# Autodesk Inventor assembly: omniwheelassmebly
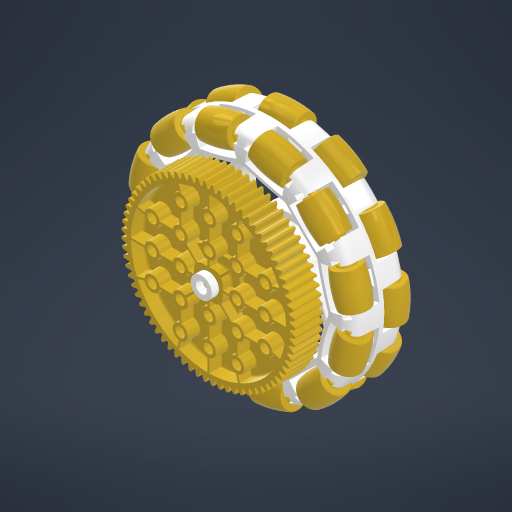
[picture p0: Inventor's stored thumbnail of the model, 512x512]
Saved by Autodesk Inventor 2023 (Build 270158000, 158)
## iProperties
Created: 2023-08-05
Part Number: omniwheelassmebly
Document SubType Name: Assembly
Designer: srbel
Author: srbel
## Documents named in this file (11)
- C:\CAD\OverUnderCAD\Drive\omniwheelassmebly.iam
- C:\CAD\OverUnderCAD\VEX-CAD-Inventor-1.4.0\Motion\Spacers\Spacer Nylon .313 OD\NSpacer .313 OD x .250.ipt
- C:\CAD\OverUnderCAD\VEX-CAD-Inventor-1.4.0\Motion\Spacers\Spacer Nylon .313 OD.ipt
- C:\CAD\OverUnderCAD\VEX-CAD-Inventor-1.4.0\Motion\Gears\HS Gear\HS 72T Gear, Square.iam
- C:\CAD\OverUnderCAD\VEX-CAD-Inventor-1.4.0\Motion\Gears\HS Gear.iam
- C:\CAD\OverUnderCAD\VEX-CAD-Inventor-1.4.0\Motion\Wheels\Omni Wheel\4 Omni, Square.iam
- C:\CAD\OverUnderCAD\VEX-CAD-Inventor-1.4.0\Motion\Wheels\Omni Wheel.iam
- C:\CAD\OverUnderCAD\VEX-CAD-Inventor-1.4.0\Motion\Spacers\Spacer Nylon .313 OD\NSpacer .313 OD x .125.ipt
- C:\CAD\OverUnderCAD\VEX-CAD-Inventor-1.4.0\Motion\Spacers\Washer Teflon\TWasher .375 OD x .04000.ipt
- C:\CAD\OverUnderCAD\VEX-CAD-Inventor-1.4.0\Motion\Spacers\Washer Teflon.ipt
- C:\CAD\OverUnderCAD\VEX-CAD-Inventor-1.4.0\Motion\Spacers\Spacer Nylon .313 OD\NSpacer .313 OD x .375.ipt
## Components (6 placed, 6 different names)
1. HS 72T Gear, Square:1 [sub-assembly] — Insert:2, Insert:7
2. NSpacer .313 OD x .250:2 — Insert:2, Insert:3
3. 4 Omni, Square:1 [sub-assembly] — Insert:3, Insert:8
4. NSpacer .313 OD x .125:4 — Insert:7
5. NSpacer .313 OD x .375:6 — Insert:8, Insert:9
6. TWasher .375 OD x .04000:2 — Insert:9
## Relationships (5: Insert 5)
- Insert:2: HS 72T Gear, Square:1 ↔ NSpacer .313 OD x .250:2
- Insert:3: NSpacer .313 OD x .250:2 ↔ 4 Omni, Square:1
- Insert:7: HS 72T Gear, Square:1 ↔ NSpacer .313 OD x .125:4
- Insert:8: 4 Omni, Square:1 ↔ NSpacer .313 OD x .375:6
- Insert:9: NSpacer .313 OD x .375:6 ↔ TWasher .375 OD x .04000:2
